# Autodesk Inventor assembly: 4inchAssemblyTest
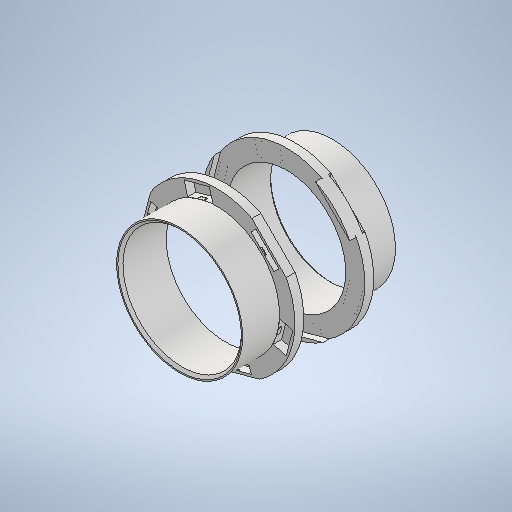
[picture p0: Inventor's stored thumbnail of the model, 512x512]
Saved by Autodesk Inventor 2025.2 (Build 292293000, 293)
## iProperties
Created: 2024-12-23
Part Number: 4inchAssemblyTest
Document SubType Name: Assembly
Designer: lidang
Author: lidang
## Documents named in this file (3)
- D:\Documents\GitRepo\3Dprinting\MagConnectionSystem\4inchAssemblyTest.iam
- D:\Documents\GitRepo\3Dprinting\MagConnectionSystem\4inchFemale.ipt
- D:\Documents\GitRepo\3Dprinting\MagConnectionSystem\4inchMale.ipt
## Components (2 placed, 2 different names)
1. 4inchFemale:1 — Mate:2, Mate:3, Mate:4, Mate:5
2. 4inchMale:1 — Mate:4, Mate:5
## Relationships (4: Mate 4)
- Mate:2: 4inchFemale:1
- Mate:3: 4inchFemale:1
- Mate:4: 4inchFemale:1 ↔ 4inchMale:1
- Mate:5: 4inchFemale:1 ↔ 4inchMale:1
